# Autodesk Inventor assembly: 下半身_6
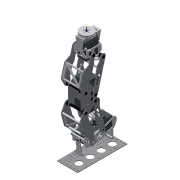
[picture p0: Inventor's stored thumbnail of the model, 180x180]
Saved by Autodesk Inventor 2016 (Build 200138000, 138)
## iProperties
Created: 2016-08-23
Part Number: 下半身_6
Material: 一般
Document SubType Name: Assembly
Designer: hiro
Mass: 908.966 g
Surface Area: 2435.97 cm^2
Volume: 423.983 cm^3
Density: 2.14387 g/cm^3
Author: hiro
## Documents named in this file (15)
- C:\Users\haya\Desktop\OpenPlatform\下半身_6.iam
- C:\Users\haya\Desktop\OpenPlatform\下半身_160823\膝\膝_6_1.iam
- C:\Users\haya\Desktop\OpenPlatform\下半身\足首\足首_1.iam
- C:\Users\haya\Desktop\OpenPlatform\下半身\足首\足首_独立ピッチ_1.iam
- C:\Users\haya\Desktop\OpenPlatform\下半身_160823\リンク\リンク_6_1.iam
- C:\Users\haya\Desktop\OpenPlatform\下半身_160823\リンク\長穴減速_ホーン_1.iam
- C:\Users\haya\Desktop\OpenPlatform\下半身_160823\リンク\リンク_6_2.iam
- C:\Users\haya\Desktop\OpenPlatform\下半身\足裏\足裏_1_1.iam
- C:\Users\haya\Desktop\OpenPlatform\下半身_160823\リンク\リンク_6_3.iam
- C:\Users\haya\Desktop\OpenPlatform\下半身_160823\リンク\長穴減速_ホーン_1_MIR.iam
- C:\Users\haya\Desktop\OpenPlatform\下半身_160823\リンク\リンク_6_4.iam
- C:\Users\haya\Desktop\OpenPlatform\下半身_160823\付け根\付け根_6_1.iam
- C:\Users\haya\Desktop\OpenPlatform\下半身_160823\付け根ロール\付け根ロール_6.iam
- C:\Users\haya\Desktop\OpenPlatform\下半身_160823\付け根ロール\長穴減速_ホーン_2.iam
- C:\Users\haya\Desktop\OpenPlatform\下半身_160823\リンク\長穴減速_ホーン_2.iam
## Components (16 placed, 13 different names)
1. 付け根ロール_6:1 [sub-assembly] — 角度:10, 角度:12, 角度:22, メイト:23, フラッシュ:25, フラッシュ:26, 角度:3, 挿入:44, 挿入:45, メイト:25
2. 膝_6_1:1 [sub-assembly] — 角度:1, 挿入:4, 挿入:15, 角度:14, 角度:15, 角度:16, 角度:17, 角度:18, 角度:19, 角度:20, 角度:21, 挿入:34, 挿入:35, 挿入:36, 挿入:37, 挿入:38, 挿入:39, 挿入:40, 挿入:41
3. 足首_1:1 [sub-assembly] — 角度:1, 挿入:11, 挿入:12, 挿入:22, 挿入:23, 挿入:28, 挿入:29, 挿入:30, 挿入:31
4. 足首_独立ピッチ_1:1 [sub-assembly] — 挿入:22, 挿入:23, 挿入:25, 挿入:24, 挿入:26, 挿入:27, 挿入:28, 挿入:29, 挿入:30, 挿入:31
5. 足裏_1_1:1 [sub-assembly] — 挿入:11, 挿入:12, 角度:3
6. 長穴減速_ホーン_1:1 [sub-assembly] — 挿入:4, 挿入:48
7. 長穴減速_ホーン_1_MIR:1 [sub-assembly] — 挿入:15, 挿入:47
8. 付け根_6_1:1 [sub-assembly] — 挿入:18, 角度:10, 角度:12, 挿入:32, 挿入:33, 挿入:42, 挿入:43, 挿入:44, 挿入:45, 角度:22
9. 長穴減速_ホーン_2:1 [sub-assembly] — 挿入:18, 挿入:46
10. リンク_6_3:1 [sub-assembly] — 挿入:32, 挿入:33, 挿入:34, 挿入:35, メイト:26
11. リンク_6_1:1 [sub-assembly] — 挿入:25, 挿入:24, 挿入:38, 挿入:39, メイト:27
12. リンク_6_4:1 [sub-assembly] — 角度:18, 角度:19, 角度:20, 角度:21, 挿入:36, 挿入:37, 挿入:42, 挿入:43
13. リンク_6_2:1 [sub-assembly] — 角度:14, 角度:15, 角度:16, 角度:17, 挿入:26, 挿入:27, 挿入:40, 挿入:41
14. 長穴減速_ホーン_2:2 [sub-assembly] — 挿入:46, メイト:25
15. 長穴減速_ホーン_2:3 [sub-assembly] — 挿入:48, メイト:27
16. 長穴減速_ホーン_2:4 [sub-assembly] — 挿入:47, メイト:26
## Relationships (51: Insert 32, Angle 13, Mate 4, Flush 2)
- 角度:1 [Angle] (0 deg): 膝_6_1:1 ↔ 足首_1:1
- 挿入:4 [Insert]: 膝_6_1:1 ↔ 長穴減速_ホーン_1:1
- 挿入:11 [Insert]: 足首_1:1 ↔ 足裏_1_1:1
- 挿入:12 [Insert]: 足首_1:1 ↔ 足裏_1_1:1
- 角度:3 [Angle] (0 deg): 付け根ロール_6:1 ↔ 足裏_1_1:1
- 挿入:15 [Insert]: 膝_6_1:1 ↔ 長穴減速_ホーン_1_MIR:1
- 挿入:18 [Insert]: 付け根_6_1:1 ↔ 長穴減速_ホーン_2:1
- 角度:10 [Angle] (-45 deg): 付け根ロール_6:1 ↔ 付け根_6_1:1
- 角度:12 [Angle] (0 deg): 付け根ロール_6:1 ↔ 付け根_6_1:1
- 角度:14 [Angle] (0 deg): 膝_6_1:1 ↔ リンク_6_2:1
- 角度:15 [Angle] (-30 deg): 膝_6_1:1 ↔ リンク_6_2:1
- 角度:16 [Angle] (15 deg): 膝_6_1:1 ↔ リンク_6_2:1
- 角度:17 [Angle] (90 deg): 膝_6_1:1 ↔ リンク_6_2:1
- 角度:18 [Angle] (0 deg): 膝_6_1:1 ↔ リンク_6_4:1
- 角度:19 [Angle] (30 deg): 膝_6_1:1 ↔ リンク_6_4:1
- 角度:20 [Angle] (-15 deg): 膝_6_1:1 ↔ リンク_6_4:1
- 角度:21 [Angle] (90 deg): 膝_6_1:1 ↔ リンク_6_4:1
- 角度:22 [Angle] (20 deg): 付け根ロール_6:1 ↔ 付け根_6_1:1
- メイト:23 [Mate]: 付け根ロール_6:1
- フラッシュ:25 [Flush]: 付け根ロール_6:1
- フラッシュ:26 [Flush]: 付け根ロール_6:1
- 挿入:22 [Insert]: 足首_1:1 ↔ 足首_独立ピッチ_1:1
- 挿入:23 [Insert]: 足首_1:1 ↔ 足首_独立ピッチ_1:1
- 挿入:26 [Insert]: 足首_独立ピッチ_1:1 ↔ リンク_6_2:1
- 挿入:27 [Insert]: 足首_独立ピッチ_1:1 ↔ リンク_6_2:1
- 挿入:28 [Insert]: 足首_1:1 ↔ 足首_独立ピッチ_1:1
- 挿入:29 [Insert]: 足首_1:1 ↔ 足首_独立ピッチ_1:1
- 挿入:30 [Insert]: 足首_1:1 ↔ 足首_独立ピッチ_1:1
- 挿入:31 [Insert]: 足首_1:1 ↔ 足首_独立ピッチ_1:1
- 挿入:32 [Insert]: 付け根_6_1:1 ↔ リンク_6_3:1
- 挿入:33 [Insert]: 付け根_6_1:1 ↔ リンク_6_3:1
- 挿入:34 [Insert]: 膝_6_1:1 ↔ リンク_6_3:1
- 挿入:35 [Insert]: 膝_6_1:1 ↔ リンク_6_3:1
- 挿入:36 [Insert]: 膝_6_1:1 ↔ リンク_6_4:1
- 挿入:37 [Insert]: 膝_6_1:1 ↔ リンク_6_4:1
- 挿入:25 [Insert]: 足首_独立ピッチ_1:1 ↔ リンク_6_1:1
- 挿入:24 [Insert]: 足首_独立ピッチ_1:1 ↔ リンク_6_1:1
- 挿入:38 [Insert]: 膝_6_1:1 ↔ リンク_6_1:1
- 挿入:39 [Insert]: 膝_6_1:1 ↔ リンク_6_1:1
- 挿入:40 [Insert]: 膝_6_1:1 ↔ リンク_6_2:1
- 挿入:41 [Insert]: 膝_6_1:1 ↔ リンク_6_2:1
- 挿入:42 [Insert]: 付け根_6_1:1 ↔ リンク_6_4:1
- 挿入:43 [Insert]: 付け根_6_1:1 ↔ リンク_6_4:1
- 挿入:44 [Insert]: 付け根ロール_6:1 ↔ 付け根_6_1:1
- 挿入:45 [Insert]: 付け根ロール_6:1 ↔ 付け根_6_1:1
- 挿入:46 [Insert]: 長穴減速_ホーン_2:1 ↔ 長穴減速_ホーン_2:2
- メイト:25 [Mate]: 付け根ロール_6:1 ↔ 長穴減速_ホーン_2:2
- 挿入:47 [Insert]: 長穴減速_ホーン_1_MIR:1 ↔ 長穴減速_ホーン_2:4
- 挿入:48 [Insert]: 長穴減速_ホーン_1:1 ↔ 長穴減速_ホーン_2:3
- メイト:26 [Mate]: リンク_6_3:1 ↔ 長穴減速_ホーン_2:4
- メイト:27 [Mate]: リンク_6_1:1 ↔ 長穴減速_ホーン_2:3
